# Autodesk Inventor assembly: новая форточка
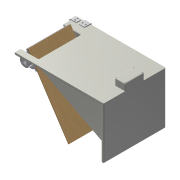
[picture p0: Inventor's stored thumbnail of the model, 180x180]
Saved by Autodesk Inventor 2021 (Build 250183000, 183)
## iProperties
Created: 2023-02-20
Part Number: новая форточка
Document SubType Name: Assembly
Designer: Tasya
Author: Tasya
## Documents named in this file (10)
- C:\Users\Tasya\Desktop\теплица\3D\Сборки iam\новая форточка.iam
- C:\Users\Tasya\Desktop\теплица\форточка\основание форточки.ipt
- C:\Users\Tasya\Desktop\теплица\форточка\servo arm.ipt
- C:\Users\Tasya\Desktop\теплица\форточка\вал форточка.ipt
- C:\Users\Tasya\Desktop\теплица\форточка\коробка + сервак.iam
- C:\Users\Tasya\Desktop\теплица\форточка\корпус подшипник.ipt
- C:\Users\Tasya\Desktop\теплица\форточка\кронштейн.ipt
- C:\Users\Tasya\Desktop\теплица\форточка\подшипник.ipt
- C:\Users\Tasya\Desktop\теплица\форточка\форточка.ipt
- C:\Users\Tasya\Desktop\теплица\grabcad\Switch on off.ipt
## Components (9 placed, 9 different names)
1. основание форточки:1 — Совмещение:1, Совмещение:2, Совмещение:3, Совмещение:12, Совмещение:13, Совмещение:14, Совмещение:16, Совмещение:17, Совмещение:18
2. servo arm:1 — Совмещение:6, Совмещение:7, Совмещение:8, Совмещение:9, Совмещение:10
3. вал форточка:1 — Совмещение:8, Совмещение:9, Совмещение:10, Совмещение:15, Заподлицо:2, Заподлицо:3
4. коробка + сервак:1 [sub-assembly] — Совмещение:4, Совмещение:5, Совмещение:6, Совмещение:7
5. корпус подшипник:1 — Совмещение:11, Заподлицо:1, Совмещение:12, Совмещение:13, Совмещение:14
6. кронштейн:1 — Совмещение:1, Совмещение:2, Совмещение:3, Совмещение:4, Совмещение:5
7. подшипник:1 — Совмещение:11, Заподлицо:1
8. форточка:1 — Совмещение:15, Заподлицо:2, Заподлицо:3
9. Switch on off:1 — Совмещение:16, Совмещение:17, Совмещение:18
## Relationships (21: Mate 18, Flush 3)
- Совмещение:1 [Mate]: основание форточки:1 ↔ кронштейн:1
- Совмещение:2 [Mate]: основание форточки:1 ↔ кронштейн:1
- Совмещение:3 [Mate]: основание форточки:1 ↔ кронштейн:1
- Совмещение:4 [Mate]: коробка + сервак:1 ↔ кронштейн:1
- Совмещение:5 [Mate]: коробка + сервак:1 ↔ кронштейн:1
- Совмещение:6 [Mate]: servo arm:1 ↔ коробка + сервак:1
- Совмещение:7 [Mate]: servo arm:1 ↔ коробка + сервак:1
- Совмещение:8 [Mate]: servo arm:1 ↔ вал форточка:1
- Совмещение:9 [Mate]: servo arm:1 ↔ вал форточка:1
- Совмещение:10 [Mate]: servo arm:1 ↔ вал форточка:1
- Совмещение:11 [Mate]: корпус подшипник:1 ↔ подшипник:1
- Заподлицо:1 [Flush]: корпус подшипник:1 ↔ подшипник:1
- Совмещение:12 [Mate]: основание форточки:1 ↔ корпус подшипник:1
- Совмещение:13 [Mate]: основание форточки:1 ↔ корпус подшипник:1
- Совмещение:14 [Mate]: основание форточки:1 ↔ корпус подшипник:1
- Совмещение:15 [Mate]: вал форточка:1 ↔ форточка:1
- Заподлицо:2 [Flush]: вал форточка:1 ↔ форточка:1
- Заподлицо:3 [Flush]: вал форточка:1 ↔ форточка:1
- Совмещение:16 [Mate]: основание форточки:1 ↔ Switch on off:1
- Совмещение:17 [Mate]: основание форточки:1 ↔ Switch on off:1
- Совмещение:18 [Mate] (1 mm): основание форточки:1 ↔ Switch on off:1
